# Autodesk Inventor assembly: test
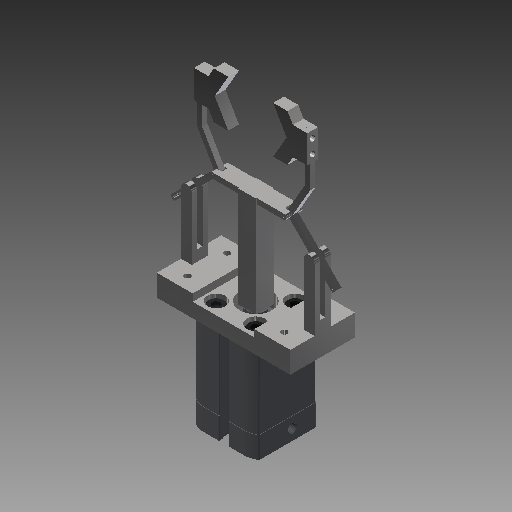
[picture p0: Inventor's stored thumbnail of the model, 512x512]
Saved by Autodesk Inventor 2017 (Build 210142000, 142)
## iProperties
Created: 2018-05-29
Part Number: test
Document SubType Name: Assembly
Designer: Pies
Author: Pies
## Documents named in this file (10)
- C:\Users\Pies\Desktop\Rzeczy\AGH\Semestr 2\ZIPK\Chwytak\Moj_Chwd_Pytak\Inventorowe chwytaki\Gotowy chwytak.iam
- C:\Users\Pies\Desktop\Rzeczy\AGH\Semestr 2\ZIPK\Chwytak\Moj_Chwd_Pytak\Inventorowe chwytaki\Ciągaczka.ipt
- C:\Users\Pies\Desktop\Rzeczy\AGH\Semestr 2\ZIPK\Chwytak\Moj_Chwd_Pytak\Inventorowe chwytaki\PIN.ipt
- C:\Users\Pies\Desktop\Rzeczy\AGH\Semestr 2\ZIPK\Chwytak\Moj_Chwd_Pytak\Inventorowe chwytaki\Ramię z łapką.iam
- C:\Users\Pies\Desktop\Rzeczy\AGH\Semestr 2\ZIPK\Chwytak\Moj_Chwd_Pytak\Inventorowe chwytaki\Podstawka.ipt
- C:\Users\Pies\Desktop\Rzeczy\AGH\Semestr 2\ZIPK\Chwytak\Moj_Chwd_Pytak\Inventorowe chwytaki\MOJ KOLNIERZ.ipt
- C:\Users\Pies\Desktop\Rzeczy\AGH\Semestr 2\ZIPK\Chwytak\Moj_Chwd_Pytak\Inventorowe chwytaki\Silownik\536236 ADN-20-15-A-P-A---(asm_0).iam
- C:\Users\Pies\Desktop\Rzeczy\AGH\Semestr 2\ZIPK\Chwytak\Moj_Chwd_Pytak\Inventorowe chwytaki\Kołnierz\DIN-6912 - M5x20(F).ipt
- C:\Users\Pies\Documents\Inventor\Content Center Files\R2017\en-US\SS-ISO 4762\ISO 4762 - M3 x 12SS-ISO.ipt
- C:\Users\Pies\Documents\Inventor\Content Center Files\R2017\en-US\SS-ISO 4762\ISO 4762 - M3 x 8SS-ISO.ipt
## Components (23 placed, 9 different names)
1. PIN:1 — Rigid:2
2. PIN:2 — Rigid:3
3. PIN:3 — Rigid:6, Tangent:2
4. PIN:4 — Rigid:5, Tangent:1
5. Ramię z łapką:1 [sub-assembly] — Rotational:1, Tangent:1, Mate:42, Mate:43, Mate:44
6. Ramię z łapką:2 [sub-assembly] — Rotational:2, Tangent:2, Mate:39, Mate:40, Mate:41
7. Ciągaczka:1 — Rotational:1, Rotational:2, Rigid:2, Rigid:3, Mate:10
8. Podstawka:1 — Rigid:5, Mate:31, Mate:32, Mate:34, Mate:37, Mate:38
9. Podstawka:2 — Rigid:6, Mate:29, Mate:30, Mate:33, Mate:35, Mate:36
10. MOJ KOLNIERZ:1 — Mate:10, Mate:19, Mate:20, Mate:23, Mate:24, Mate:25, Mate:26, Mate:28, Mate:29, Mate:30, Mate:31, Mate:32, Mate:33, Mate:34
11. 536236 ADN-20-15-A-P-A---(asm_0):1 [sub-assembly] — Mate:26, Mate:27, Mate:28
12. DIN-6912 - M5x20(F):1 — Mate:19
13. DIN-6912 - M5x20(F):2 — Mate:20
14. DIN-6912 - M5x20(F):3 — Mate:25, Mate:27
15. DIN-6912 - M5x20(F):4 — Mate:23, Mate:24
16. SS ISO 4762 M3 x 12:1 — Mate:35
17. SS ISO 4762 M3 x 12:2 — Mate:36
18. SS ISO 4762 M3 x 12:3 — Mate:37
19. SS ISO 4762 M3 x 12:4 — Mate:38
20. SS ISO 4762 M3 x 8:1 — Mate:39, Mate:40
21. SS ISO 4762 M3 x 8:2 — Mate:41
22. SS ISO 4762 M3 x 8:3 — Mate:42, Mate:43
23. SS ISO 4762 M3 x 8:4 — Mate:44
## Relationships (33: Mate 25, WeldJoint 4, RevoluteJoint 2, Tangent 2)
- Rotational:1 [RevoluteJoint]: Ramię z łapką:1 ↔ Ciągaczka:1
- Rotational:2 [RevoluteJoint]: Ramię z łapką:2 ↔ Ciągaczka:1
- Rigid:2 [WeldJoint]: PIN:1 ↔ Ciągaczka:1
- Rigid:3 [WeldJoint]: PIN:2 ↔ Ciągaczka:1
- Mate:10: Ciągaczka:1 ↔ MOJ KOLNIERZ:1
- Rigid:5 [WeldJoint]: PIN:4 ↔ Podstawka:1
- Mate:19: MOJ KOLNIERZ:1 ↔ DIN-6912 - M5x20(F):1
- Mate:20: MOJ KOLNIERZ:1 ↔ DIN-6912 - M5x20(F):2
- Mate:23: MOJ KOLNIERZ:1 ↔ DIN-6912 - M5x20(F):4
- Mate:24: MOJ KOLNIERZ:1 ↔ DIN-6912 - M5x20(F):4
- Mate:25: MOJ KOLNIERZ:1 ↔ DIN-6912 - M5x20(F):3
- Mate:26: MOJ KOLNIERZ:1 ↔ 536236 ADN-20-15-A-P-A---(asm_0):1
- Mate:27: 536236 ADN-20-15-A-P-A---(asm_0):1 ↔ DIN-6912 - M5x20(F):3
- Mate:28: MOJ KOLNIERZ:1 ↔ 536236 ADN-20-15-A-P-A---(asm_0):1
- Rigid:6 [WeldJoint]: PIN:3 ↔ Podstawka:2
- Mate:29: Podstawka:2 ↔ MOJ KOLNIERZ:1
- Mate:30: Podstawka:2 ↔ MOJ KOLNIERZ:1
- Mate:31: Podstawka:1 ↔ MOJ KOLNIERZ:1
- Mate:32: Podstawka:1 ↔ MOJ KOLNIERZ:1
- Mate:33: Podstawka:2 ↔ MOJ KOLNIERZ:1
- Mate:34: Podstawka:1 ↔ MOJ KOLNIERZ:1
- Tangent:1: PIN:4 ↔ Ramię z łapką:1
- Tangent:2: PIN:3 ↔ Ramię z łapką:2
- Mate:35: Podstawka:2 ↔ SS ISO 4762 M3 x 12:1
- Mate:36: Podstawka:2 ↔ SS ISO 4762 M3 x 12:2
- Mate:37: Podstawka:1 ↔ SS ISO 4762 M3 x 12:3
- Mate:38: Podstawka:1 ↔ SS ISO 4762 M3 x 12:4
- Mate:39: Ramię z łapką:2 ↔ SS ISO 4762 M3 x 8:1
- Mate:40: Ramię z łapką:2 ↔ SS ISO 4762 M3 x 8:1
- Mate:41: Ramię z łapką:2 ↔ SS ISO 4762 M3 x 8:2
- Mate:42: Ramię z łapką:1 ↔ SS ISO 4762 M3 x 8:3
- Mate:43: Ramię z łapką:1 ↔ SS ISO 4762 M3 x 8:3
- Mate:44: Ramię z łapką:1 ↔ SS ISO 4762 M3 x 8:4
